# Autodesk Inventor assembly: torso
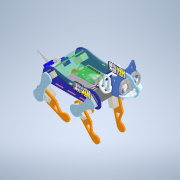
[picture p0: Inventor's stored thumbnail of the model, 180x180]
Saved by Autodesk Inventor 2020.3 (Build 243373000, 373)
## iProperties
Created: 2020-08-06
Part Number: torso
Document SubType Name: Assembly
Designer: aditk
Author: aditk
## Documents named in this file (18)
- C:\Users\aditk\Desktop\PETcat\newCat\torso.iam
- C:\Users\aditk\Desktop\PETcat\newCat\torso_base.ipt
- C:\Users\aditk\Desktop\PETcat\newCat\torso side.ipt
- C:\Users\aditk\Desktop\PETcat\newCat\sholder.ipt
- C:\Users\aditk\Desktop\PETcat\newCat\tail.ipt
- C:\Users\aditk\Desktop\PETcat\newCat\head.ipt
- C:\Users\aditk\Desktop\PETcat\newCat\big_servo.ipt
- C:\Users\aditk\Desktop\PETcat\newCat\LEG1.iam
- C:\Users\aditk\Desktop\PETcat\newCat\LEG2.iam
- C:\Users\aditk\Desktop\PETcat\newCat\PETcat\withsensors\16-channel-pwm-servo-controller-1.snapshot.2\Arduino 16 Channel PWM Module\12Channel PWM.ipt
- C:\Users\aditk\Desktop\PETcat\newCat\PETcat\withsensors\raspberry-pi-4-b-work-in-progress-1.snapshot.6\Raspberry Pi 4 B.ipt
- C:\Users\aditk\Desktop\PETcat\newCat\PETcat\withsensors\mpu-9250-9dof-imu-1.snapshot.4\MPU-9250.iam
- C:\Users\aditk\Desktop\PETcat\newCat\PETcat\withsensors\User Library-OV2640\User Library-OV2640.ipt
- C:\Users\aditk\Desktop\PETcat\newCat\hook.ipt
- C:\Users\aditk\Desktop\PETcat\newCat\hook_MIR.ipt
- C:\Users\aditk\Desktop\PETcat\newCat\cover.ipt
- C:\Users\aditk\Desktop\PETcat\newCat\clip.ipt
- C:\Users\aditk\Desktop\PETcat\newCat\tail_end.ipt
## Components (35 placed, 18 different names)
1. torso_base:1 — Mate:1, Mate:2, Mate:3, Mate:4, Mate:5, Mate:6, Mate:7, Mate:32, Mate:33, Mate:34
2. torso side:1 — Mate:2, Mate:3, Mate:4, Mate:8, Mate:9, Mate:10, Mate:20, Mate:21, Mate:28, Mate:29, Mate:30, Mate:31, Insert:9, Insert:10, Insert:11, Insert:12, Symmetry:1, Mate:36, Mate:37
3. torso side:2 — Mate:5, Mate:6, Mate:7, Mate:11, Mate:12, Mate:13, Mate:22, Mate:23, Mate:24, Mate:25, Mate:26, Mate:27, Symmetry:1, Mate:35
4. sholder:1 — Mate:9, Mate:11, Mate:12, Mate:17, Mate:18, Mate:19
5. sholder:2 — Mate:8, Mate:10, Mate:13, Mate:14, Mate:15, Mate:16
6. small_servo:1 [sub-assembly] — Mate:14, Mate:15, Mate:16, Insert:13
7. small_servo:2 [sub-assembly] — Mate:17, Mate:18, Mate:19, Insert:2
8. tail:1 — Insert:13, Insert:14, Insert:15
9. head:1 — Insert:2, Insert:7, Insert:8
10. big_servo:1 — Mate:20, Mate:28, Mate:29, Insert:6
11. big_servo:2 — Mate:21, Mate:30, Mate:31, Insert:5
12. big_servo:3 — Mate:22, Mate:25, Mate:26, Insert:3
13. big_servo:4 — Mate:23, Mate:24, Mate:27, Insert:4
14. LEG1:1 [sub-assembly] — Insert:4
15. LEG1:2 [sub-assembly] — Insert:3
16. LEG2:1 [sub-assembly] — Insert:5
17. LEG2:2 [sub-assembly] — Insert:6
18. 12Channel PWM:1 — Mate:34
19. Raspberry Pi 4 B:1 — Mate:32
20. MPU-9250:1 [sub-assembly] — Mate:33
21. User Library-OV2640:1 — Insert:8
22. User Library-OV2640:2 — Insert:7
23. hook:1 — Insert:12
24. hook:2 — Insert:11
25. hook:3 — Insert:10
26. hook:4 — Insert:9
27. hook_MIR:1
28. hook_MIR:2
29. hook_MIR:3
30. hook_MIR:4
31. cover:1 — Mate:35, Mate:36, Mate:37, Mate:38, Mate:39, Mate:40, Mate:41, Mate:42, Mate:43
32. clip:1 — Mate:38, Mate:39, Mate:40
33. clip:2 — Mate:41, Mate:42, Mate:43
34. tail_end:1 — Insert:16
35. small_servo:3 [sub-assembly] — Insert:14, Insert:15, Insert:16
## Relationships (59: Mate 43, Insert 15, Symmetry 1)
- Mate:1: torso_base:1
- Mate:2: torso_base:1 ↔ torso side:1
- Mate:3: torso_base:1 ↔ torso side:1
- Mate:4: torso_base:1 ↔ torso side:1
- Mate:5: torso_base:1 ↔ torso side:2
- Mate:6: torso_base:1 ↔ torso side:2
- Mate:7: torso_base:1 ↔ torso side:2
- Mate:8: torso side:1 ↔ sholder:2
- Mate:9: torso side:1 ↔ sholder:1
- Mate:10: torso side:1 ↔ sholder:2
- Mate:11: torso side:2 ↔ sholder:1
- Mate:12: torso side:2 ↔ sholder:1
- Mate:13: torso side:2 ↔ sholder:2
- Mate:14: sholder:2 ↔ small_servo:1
- Mate:15: sholder:2 ↔ small_servo:1
- Mate:16: sholder:2 ↔ small_servo:1
- Mate:17: sholder:1 ↔ small_servo:2
- Mate:18: sholder:1 ↔ small_servo:2
- Mate:19: sholder:1 ↔ small_servo:2
- Insert:2: small_servo:2 ↔ head:1
- Mate:20: torso side:1 ↔ big_servo:1
- Mate:21: torso side:1 ↔ big_servo:2
- Mate:22: torso side:2 ↔ big_servo:3
- Mate:23: torso side:2 ↔ big_servo:4
- Mate:24: torso side:2 ↔ big_servo:4
- Mate:25: torso side:2 ↔ big_servo:3
- Mate:26: torso side:2 ↔ big_servo:3
- Mate:27: torso side:2 ↔ big_servo:4
- Mate:28: torso side:1 ↔ big_servo:1
- Mate:29: torso side:1 ↔ big_servo:1
- Mate:30: torso side:1 ↔ big_servo:2
- Mate:31: torso side:1 ↔ big_servo:2
- Insert:3 (0.1 mm): big_servo:3 ↔ LEG1:2
- Insert:4 (0.1 mm): big_servo:4 ↔ LEG1:1
- Insert:5 (0.1 mm): big_servo:2 ↔ LEG2:1
- Insert:6 (0.1 mm): big_servo:1 ↔ LEG2:2
- Mate:32 (3 mm): torso_base:1 ↔ Raspberry Pi 4 B:1
- Mate:33 (10 mm): torso_base:1 ↔ MPU-9250:1
- Mate:34 (3 mm): torso_base:1 ↔ 12Channel PWM:1
- Insert:7: head:1 ↔ User Library-OV2640:2
- Insert:8: head:1 ↔ User Library-OV2640:1
- Insert:9 (0.01 mm): torso side:1 ↔ hook:4
- Insert:10: torso side:1 ↔ hook:3
- Insert:11: torso side:1 ↔ hook:2
- Insert:12: torso side:1 ↔ hook:1
- Symmetry:1: torso side:1 ↔ torso side:2
- Mate:35: torso side:2 ↔ cover:1
- Mate:36: torso side:1 ↔ cover:1
- Mate:37: torso side:1 ↔ cover:1
- Mate:38: cover:1 ↔ clip:1
- Mate:39: cover:1 ↔ clip:1
- Mate:40: cover:1 ↔ clip:1
- Mate:41: cover:1 ↔ clip:2
- Mate:42: cover:1 ↔ clip:2
- Mate:43: cover:1 ↔ clip:2
- Insert:13: small_servo:1 ↔ tail:1
- Insert:14: tail:1 ↔ small_servo:3
- Insert:15: tail:1 ↔ small_servo:3
- Insert:16: tail_end:1 ↔ small_servo:3
